# Autodesk Inventor assembly: mascon-new
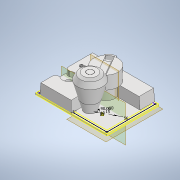
[picture p0: Inventor's stored thumbnail of the model, 180x180]
Saved by Autodesk Inventor 2021 (Build 250183000, 183)
## iProperties
Created: 2021-04-28
Part Number: mascon-new
Document SubType Name: Assembly
Designer: ben
Author: ben
## Documents named in this file (5)
- C:\Users\teh18\OneDrive\BVE Controller\r68-bve-mascon\mascon-new.iam
- C:\Users\teh18\OneDrive\BVE Controller\r68-bve-mascon\mascon.ipt
- C:\Users\teh18\OneDrive\BVE Controller\r68-bve-mascon\handle_base2.ipt
- C:\Users\teh18\OneDrive\BVE Controller\r68-bve-mascon\handle-base\handle-base.iam
- C:\Users\teh18\OneDrive\BVE Controller\r68-bve-mascon\handle\handle.iam
## Components (4 placed, 4 different names)
1. mascon:1 — Mate:8, Mate:9, handle turn
2. handle_base2:1 — Mate:10, Mate:11, Mate:12
3. handle-base:1 [sub-assembly] — Mate:8, Mate:9, handle turn, Mate:10, Mate:11, Mate:12, handle pop
4. handle:1 [sub-assembly] — handle pop
## Relationships (7: Mate 5, RevoluteJoint 2)
- Mate:8: mascon:1 ↔ handle-base:1
- Mate:9: mascon:1 ↔ handle-base:1
- handle turn [RevoluteJoint]: mascon:1 ↔ handle-base:1
- Mate:10: handle_base2:1 ↔ handle-base:1
- Mate:11: handle_base2:1 ↔ handle-base:1
- Mate:12: handle_base2:1 ↔ handle-base:1
- handle pop [RevoluteJoint]: handle-base:1 ↔ handle:1
